# Autodesk Inventor assembly: Assembly_XYTable_Alexpress_75_55mm
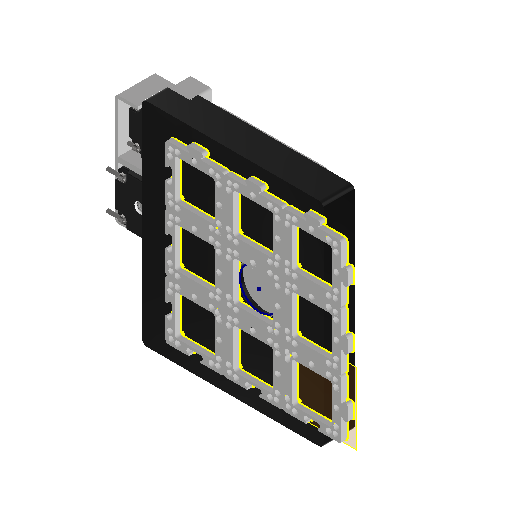
[picture p0: Inventor's stored thumbnail of the model, 512x512]
Saved by Autodesk Inventor 2023 (Build 270158000, 158)
## iProperties
Created: 2022-06-02
Part Number: Assembly_XYTable_Alexpress_75_55mm
Document SubType Name: Assembly
Designer: diederichbenedict
Author: diederichbenedict
## Documents named in this file (12)
- C:\Users\diederichbenedict\Downloads\UC2 setup design\UC2 setup design\Assembly_XYTable_Alexpress_75_55mm.iam
- C:\Users\diederichbenedict\Downloads\UC2 setup design\UC2 setup design\00_XYTable_china_75_55mm.ipt
- C:\Users\diederichbenedict\Downloads\UC2 setup design\UC2 setup design\30_XYTabel_Aliexpress_basplateadapter.ipt
- C:\Users\diederichbenedict\Downloads\UC2 setup design\UC2 setup design\30_XYTable_Aliexpress_motormount.ipt
- C:\Users\diederichbenedict\Downloads\UC2 setup design\UC2 setup design\30_XYTable_Aliexpress_sampleinsert_round.ipt
- C:\Users\diederichbenedict\Downloads\UC2 setup design\UC2 setup design\SMLM_Holder_v1.iam
- C:\Users\diederichbenedict\Downloads\UC2 setup design\UC2 setup design\00_NEMA17_pancake.iam
- C:\Users\diederichbenedict\Downloads\UC2 setup design\UC2 setup design\00_XYTable_pulley.ipt
- C:\Users\diederichbenedict\Downloads\UC2 setup design\UC2 setup design\00_XYTable_medium_gear.ipt
- C:\Users\diederichbenedict\Downloads\UC2 setup design\UC2 setup design\00_XYTable_large_gear.ipt
- C:\Users\diederichbenedict\Downloads\UC2 setup design\UC2 setup design\00_GT2_TimingBelt_flexible_Modular_xytable_large_89tooth.ipt
- C:\Users\diederichbenedict\Downloads\UC2 setup design\UC2 setup design\00_GT2_TimingBelt_flexible_Modular_xytable_large_65tooth.ipt
## Components (13 placed, 11 different names)
1. 00_XYTable_china_75_55mm:1 — Passend:1, Passend:2, Winkel:3, Passend:3, Fluchtend:1, Fluchtend:2, Passend:4, Passend:5, Passend:6, Einfügen:7
2. 30_XYTabel_Aliexpress_basplateadapter:1 — Passend:1, Passend:2, Winkel:3
3. 30_XYTable_Aliexpress_motormount:1 — Passend:3, Fluchtend:1, Fluchtend:2
4. 30_XYTable_Aliexpress_sampleinsert_round:1 — Passend:4, Passend:5, Passend:6, Einfügen:4
5. SMLM_Holder_v1:1 [sub-assembly] — Einfügen:4
6. 00_NEMA17_pancake:1 [sub-assembly] — Einfügen:6
7. 00_NEMA17_pancake:2 [sub-assembly] — Einfügen:5
8. 00_XYTable_pulley:1 — Einfügen:5, Mate:7, Mate:8
9. 00_XYTable_pulley:2 — Einfügen:6, Mate:9
10. 00_XYTable_medium_gear:1 — Einfügen:8
11. 00_XYTable_large_gear:1 — Einfügen:7, Einfügen:8
12. 00_GT2_TimingBelt_flexible_Modular_xytable_large_65tooth:1 — Mate:9
13. 00_GT2_TimingBelt_flexible_Modular_xytable_large_89tooth:1 — Mate:7, Mate:8
## Relationships (22: Mate 9, Insert 8, Angle 3, Flush 2)
- [Insert]: 30_XYTable_Aliexpress_sampleinsert_round:1 ↔ SMLM_Holder_v1:1
- [Insert]: 30_XYTable_Aliexpress_motormount:1 ↔ 00_NEMA17_pancake:1
- [Angle] (0 deg): 30_XYTable_Aliexpress_motormount:1 ↔ 00_NEMA17_pancake:1
- [Insert]: 30_XYTable_Aliexpress_motormount:1 ↔ 00_NEMA17_pancake:2
- [Angle] (0 deg): 30_XYTable_Aliexpress_motormount:1 ↔ 00_NEMA17_pancake:2
- Passend:1 [Mate]: 00_XYTable_china_75_55mm:1 ↔ 30_XYTabel_Aliexpress_basplateadapter:1
- Passend:2 [Mate]: 00_XYTable_china_75_55mm:1 ↔ 30_XYTabel_Aliexpress_basplateadapter:1
- Winkel:3 [Angle] (0 deg): 00_XYTable_china_75_55mm:1 ↔ 30_XYTabel_Aliexpress_basplateadapter:1
- Passend:3 [Mate]: 00_XYTable_china_75_55mm:1 ↔ 30_XYTable_Aliexpress_motormount:1
- Fluchtend:1 [Flush]: 00_XYTable_china_75_55mm:1 ↔ 30_XYTable_Aliexpress_motormount:1
- Fluchtend:2 [Flush] (3 mm): 00_XYTable_china_75_55mm:1 ↔ 30_XYTable_Aliexpress_motormount:1
- Passend:4 [Mate]: 00_XYTable_china_75_55mm:1 ↔ 30_XYTable_Aliexpress_sampleinsert_round:1
- Passend:5 [Mate]: 00_XYTable_china_75_55mm:1 ↔ 30_XYTable_Aliexpress_sampleinsert_round:1
- Passend:6 [Mate]: 00_XYTable_china_75_55mm:1 ↔ 30_XYTable_Aliexpress_sampleinsert_round:1
- Einfügen:4 [Insert]: 30_XYTable_Aliexpress_sampleinsert_round:1 ↔ SMLM_Holder_v1:1
- Einfügen:5 [Insert]: 00_NEMA17_pancake:2 ↔ 00_XYTable_pulley:1
- Einfügen:6 [Insert]: 00_NEMA17_pancake:1 ↔ 00_XYTable_pulley:2
- Einfügen:7 [Insert]: 00_XYTable_china_75_55mm:1 ↔ 00_XYTable_large_gear:1
- Einfügen:8 [Insert]: 00_XYTable_medium_gear:1 ↔ 00_XYTable_large_gear:1
- Mate:7 (20 mm): 00_XYTable_pulley:1 ↔ 00_GT2_TimingBelt_flexible_Modular_xytable_large_89tooth:1
- Mate:8 (10 mm): 00_XYTable_pulley:1 ↔ 00_GT2_TimingBelt_flexible_Modular_xytable_large_89tooth:1
- Mate:9 (10 mm): 00_XYTable_pulley:2 ↔ 00_GT2_TimingBelt_flexible_Modular_xytable_large_65tooth:1
